# Autodesk Inventor assembly: Fr.wing2
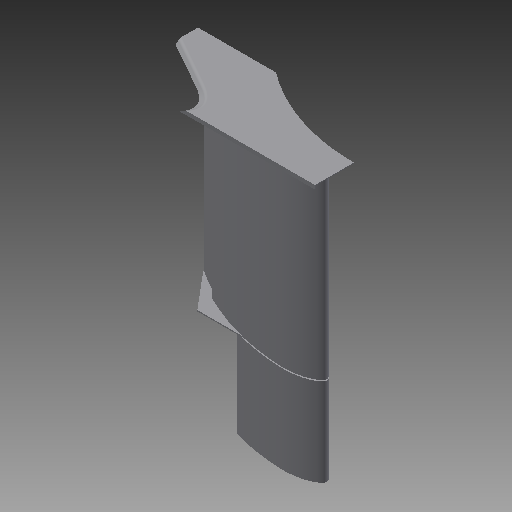
[picture p0: Inventor's stored thumbnail of the model, 512x512]
Saved by Autodesk Inventor 2018.2 (Build 222227000, 227)
## iProperties
Created: 2018-02-26
Part Number: Fr.wing2
Material: 一般
Document SubType Name: Assembly
Designer: ku_sk
Author: ku_sk
## Documents named in this file (7)
- C:\Users\ku_sk\Documents\Inventor\AeroCAD2018\設計\Fr.wing\Fr.wing2.iam
- C:\Users\ku_sk\Documents\Inventor\AeroCAD2018\設計\Fr.wing\parts\endplate3.ipt
- C:\Users\ku_sk\Documents\Inventor\AeroCAD2018\設計\Fr.wing\parts\mainflap3.ipt
- C:\Users\ku_sk\Documents\Inventor\AeroCAD2018\設計\Fr.wing\parts\subflap4.ipt
- C:\Users\ku_sk\Documents\Inventor\AeroCAD2018\設計\Fr.wing\parts\subflap23.ipt
- C:\Users\ku_sk\Documents\Inventor\AeroCAD2018\設計\Fr.wing\parts\bracket3.ipt
- C:\Users\ku_sk\Documents\Inventor\AeroCAD2018\設計\Fr.wing\parts\mainflapcenter3.ipt
## Components (6 placed, 6 different names)
1. endplate3:1 — メイト:1, メイト:2, メイト:4, メイト:5
2. mainflap3:1 — メイト:2, 角度:1, メイト:6, メイト:8
3. subflap4:1 — メイト:4, 角度:2
4. subflap23:1 — 角度:2, 角度:1, メイト:5
5. bracket3:1 — メイト:6, メイト:7
6. mainflapcenter3:1 — メイト:8, メイト:7
## Relationships (9: Mate 6, Angle 2, Flush 1)
- メイト:1 [Flush]: endplate3:1
- メイト:2 [Mate]: endplate3:1 ↔ mainflap3:1
- メイト:4 [Mate]: endplate3:1 ↔ subflap4:1
- 角度:2 [Angle] (-15 deg): subflap4:1 ↔ subflap23:1
- 角度:1 [Angle] (-15 deg): mainflap3:1 ↔ subflap23:1
- メイト:5 [Mate]: endplate3:1 ↔ subflap23:1
- メイト:6 [Mate]: mainflap3:1 ↔ bracket3:1
- メイト:8 [Mate]: mainflap3:1 ↔ mainflapcenter3:1
- メイト:7 [Mate]: bracket3:1 ↔ mainflapcenter3:1
